# Autodesk Inventor assembly: BRIDA DE APRIETE COMPLETA
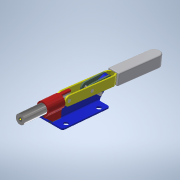
[picture p0: Inventor's stored thumbnail of the model, 180x180]
Saved by Autodesk Inventor 2021 (Build 250183000, 183)
## iProperties
Created: 2018-10-25
Part Number: BRIDA DE APRIETE COMPLETA
Document SubType Name: Assembly
Designer: Isaac
Author: Isaac
## Documents named in this file (13)
- E:\Users\Almanzor\Documents\Escuela\LABORATORIO DISEÑO Y MANUFACTURA ASISTIDA POR COMPUTADORA\Practica 8\BRIDA DE APRIETE\BRIDA DE APRIETE\BRIDA DE APRIETE COMPLETA.iam
- E:\Users\Almanzor\Documents\Escuela\LABORATORIO DISEÑO Y MANUFACTURA ASISTIDA POR COMPUTADORA\Practica 8\BRIDA DE APRIETE\BRIDA DE APRIETE\Assembly_BRIDA.iam
- E:\Users\Almanzor\Documents\Escuela\LABORATORIO DISEÑO Y MANUFACTURA ASISTIDA POR COMPUTADORA\Practica 8\BRIDA DE APRIETE\BRIDA DE APRIETE\Part4_PASADOR17.2.ipt
- E:\Users\Almanzor\Documents\Escuela\LABORATORIO DISEÑO Y MANUFACTURA ASISTIDA POR COMPUTADORA\Practica 8\BRIDA DE APRIETE\BRIDA DE APRIETE\Part3.ipt
- E:\Users\Almanzor\Documents\Escuela\LABORATORIO DISEÑO Y MANUFACTURA ASISTIDA POR COMPUTADORA\Practica 8\BRIDA DE APRIETE\BRIDA DE APRIETE\PIEZA4_COMPLETA.iam
- E:\Users\Almanzor\Documents\Escuela\LABORATORIO DISEÑO Y MANUFACTURA ASISTIDA POR COMPUTADORA\Practica 8\BRIDA DE APRIETE\BRIDA DE APRIETE\Part5.ipt
- E:\Users\Almanzor\Documents\Escuela\LABORATORIO DISEÑO Y MANUFACTURA ASISTIDA POR COMPUTADORA\Practica 8\BRIDA DE APRIETE\BRIDA DE APRIETE\Part5_GOMA.ipt
- E:\Users\Almanzor\Documents\Escuela\LABORATORIO DISEÑO Y MANUFACTURA ASISTIDA POR COMPUTADORA\Practica 8\BRIDA DE APRIETE\BRIDA DE APRIETE\BRIDA DE APRIETE COMPLETA\AIP\FEA\d6z4grx34.fins
- E:\Users\Almanzor\Documents\Escuela\LABORATORIO DISEÑO Y MANUFACTURA ASISTIDA POR COMPUTADORA\Practica 8\BRIDA DE APRIETE\BRIDA DE APRIETE\BRIDA DE APRIETE COMPLETA\AIP\FEA\d6z4grx34.fsat
- E:\Users\Almanzor\Documents\Escuela\LABORATORIO DISEÑO Y MANUFACTURA ASISTIDA POR COMPUTADORA\Practica 8\BRIDA DE APRIETE\BRIDA DE APRIETE\BRIDA DE APRIETE COMPLETA\AIP\FEA\d6z4grx34.ftes
- E:\Users\Almanzor\Documents\Escuela\LABORATORIO DISEÑO Y MANUFACTURA ASISTIDA POR COMPUTADORA\Practica 8\BRIDA DE APRIETE\BRIDA DE APRIETE\BRIDA DE APRIETE COMPLETA\AIP\FEA\d6z4grx34.fwiz
- E:\Users\Almanzor\Documents\Escuela\LABORATORIO DISEÑO Y MANUFACTURA ASISTIDA POR COMPUTADORA\Practica 8\BRIDA DE APRIETE\BRIDA DE APRIETE\BRIDA DE APRIETE COMPLETA\AIP\FEA\d6z4grxb4.fmsh
- E:\Users\Almanzor\Documents\Escuela\LABORATORIO DISEÑO Y MANUFACTURA ASISTIDA POR COMPUTADORA\Practica 8\BRIDA DE APRIETE\BRIDA DE APRIETE\BRIDA DE APRIETE COMPLETA\AIP\FEA\d6z86kppc.fres
## Components (7 placed, 6 different names)
1. Assembly_BRIDA:1 [sub-assembly] — Mate:1, Flush:1, Mate:2, Insert:1, Ángulo:1
2. Part4_PASADOR17.2:1 — Mate:1, Flush:1
3. Part3:1 — Mate:2, Mate:3
4. PIEZA4_COMPLETA:1 [sub-assembly] — Insert:1, Insert:2, Ángulo:1
5. Part5:1 — Insert:2, Mate:3, Insert:3, Mate:4, Mate:5, Mate:6
6. Part4_PASADOR17.2:2 — Insert:3
7. Part5_GOMA:1 — Mate:4, Mate:5, Mate:6
## Relationships (11: Mate 6, Insert 3, Flush 1, Angle 1)
- Mate:1: Assembly_BRIDA:1 ↔ Part4_PASADOR17.2:1
- Flush:1 (-6.1 mm): Assembly_BRIDA:1 ↔ Part4_PASADOR17.2:1
- Mate:2: Assembly_BRIDA:1 ↔ Part3:1
- Insert:1 (1 mm): Assembly_BRIDA:1 ↔ PIEZA4_COMPLETA:1
- Insert:2: PIEZA4_COMPLETA:1 ↔ Part5:1
- Mate:3: Part3:1 ↔ Part5:1
- Insert:3: Part5:1 ↔ Part4_PASADOR17.2:2
- Mate:4: Part5:1 ↔ Part5_GOMA:1
- Mate:5: Part5:1 ↔ Part5_GOMA:1
- Mate:6: Part5:1 ↔ Part5_GOMA:1
- Ángulo:1 [Angle] (29.35 deg): Assembly_BRIDA:1 ↔ PIEZA4_COMPLETA:1
## Named parameters: sa_0 = 0, sa_1 = -9810, sa_2 = 0
note: some values were not read from the file. Shown as the stored number, unit unknown: "sa_0", "sa_1", "sa_2".
